# Autodesk Inventor assembly: Driving system
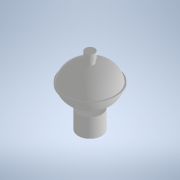
[picture p0: Inventor's stored thumbnail of the model, 180x180]
Saved by Autodesk Inventor 2020 (Build 240168000, 168)
## iProperties
Created: 2021-02-01
Part Number: Driving system
Document SubType Name: Assembly
Designer: kishore.balu
Description: Coupliing System
Engineer: LOKESH BABU/SRI SAI
Author: kishore.balu
Title: MABS-N
## Documents named in this file (4)
- C:\Users\kishore.balu\Documents\LK\New folder\New folder\Driving system.iam
- C:\Users\kishore.balu\Documents\LK\New folder\coupling_sheel.ipt
- C:\Users\kishore.balu\Documents\LK\New folder\New folder\coupling_shaft3.ipt
- C:\Users\kishore.balu\Documents\LK\New folder\coupling_shaft.ipt
## Components (4 placed, 3 different names)
1. coupling_sheel:1 — Mate:1, Mate:2, Mate:5, Mate:6
2. coupling_sheel:2 — Mate:1, Mate:2, Mate:3, Mate:4
3. coupling_shaft3:1 — Mate:3, Mate:4
4. coupling_shaft:1 — Mate:5, Mate:6
## Relationships (6: Mate 6)
- Mate:1: coupling_sheel:1 ↔ coupling_sheel:2
- Mate:2: coupling_sheel:1 ↔ coupling_sheel:2
- Mate:3: coupling_sheel:2 ↔ coupling_shaft3:1
- Mate:4: coupling_sheel:2 ↔ coupling_shaft3:1
- Mate:5: coupling_sheel:1 ↔ coupling_shaft:1
- Mate:6: coupling_sheel:1 ↔ coupling_shaft:1
